# Autodesk Inventor assembly: bed
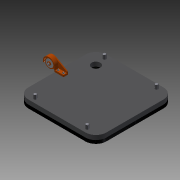
[picture p0: Inventor's stored thumbnail of the model, 180x180]
Saved by Autodesk Inventor 2013 (Build 170138000, 138)
## iProperties
Created: 2013-10-14
Part Number: bed
Document SubType Name: Assembly
Designer: employee
Author: employee
## Documents named in this file (13)
- C:\Users\employee\Desktop\ConceptFORGE\ConceptFORGE\Wally\bed.iam
- C:\Users\employee\Desktop\ConceptFORGE\ConceptFORGE\Wally\bed.ipt
- C:\Users\employee\Desktop\ConceptFORGE\ConceptFORGE\Wally\hot bed.ipt
- C:\Users\employee\Desktop\ConceptFORGE\ConceptFORGE\Wally\M3x16.ipt
- C:\Users\employee\Desktop\ConceptFORGE\ConceptFORGE\Wally\z pulley holder.ipt
- C:\Users\employee\Desktop\ConceptFORGE\ConceptFORGE\Wally\m3 nut.ipt
- C:\Users\employee\Desktop\ConceptFORGE\ConceptFORGE\Wally\608.ipt
- C:\Users\employee\Desktop\ConceptFORGE\ConceptFORGE\Wally\basalt.ipt
- C:\Users\employee\Desktop\ConceptFORGE\ConceptFORGE\Wally\M8x35.ipt
- C:\Users\employee\Desktop\ConceptFORGE\ConceptFORGE\Wally\plastic washer.ipt
- C:\Users\employee\Desktop\ConceptFORGE\ConceptFORGE\Wally\z idler.ipt
- C:\Users\employee\Desktop\ConceptFORGE\ConceptFORGE\Wally\z idler insert.ipt
- C:\Users\employee\Desktop\ConceptFORGE\ConceptFORGE\Wally\M3x14.ipt
## Components (21 placed, 11 different names)
1. bed:1 — Insert:1, Insert:2, Insert:3, Insert:11, Insert:12, Insert:22, Insert:23
2. hot bed:1 — Insert:3
3. Forged Socket Head Cap Screw - Metric M3x0.5 x 16:1 — Insert:1
4. Forged Socket Head Cap Screw - Metric M3x0.5 x 16:2 — Insert:2
5. z pulley holder:1 — Insert:22, Insert:23, Mate:1, Mate:2, Angle:1, Mate:3
6. Hex Nut Metric M3 x 0.5:1
7. Hex Nut Metric M3 x 0.5:2
8. Hex Nut Metric M3 x 0.5:3 — Mate:1, Mate:2, Angle:1
9. 608:1 — Insert:21, Mate:3, Insert:24
10. basalt:1 — Insert:11, Insert:12, Insert:13, Insert:14, Insert:15, Insert:16
11. Hex Bolt - Metric M8 x 1.25 x 35:1 — Insert:20
12. Hex Bolt - Metric M8 x 1.25 x 35:2 — Insert:19
13. Hex Bolt - Metric M8 x 1.25 x 35:3 — Insert:18
14. Hex Bolt - Metric M8 x 1.25 x 35:4 — Insert:17
15. plastic washer:1 — Insert:13, Insert:19
16. plastic washer:2 — Insert:14, Insert:18
17. plastic washer:3 — Insert:15, Insert:20
18. plastic washer:4 — Insert:16, Insert:17
19. z idler:1 — Insert:21
20. z idler insert:1 — Insert:24, Insert:25
21. Forged Socket Head Cap Screw - Metric M3x0.5 x 16:3 — Insert:25
## Relationships (22: Insert 18, Mate 3, Angle 1)
- Insert:1: bed:1 ↔ Forged Socket Head Cap Screw - Metric M3x0.5 x 16:1
- Insert:2: bed:1 ↔ Forged Socket Head Cap Screw - Metric M3x0.5 x 16:2
- Insert:3: bed:1 ↔ hot bed:1
- Insert:11: bed:1 ↔ basalt:1
- Insert:12: bed:1 ↔ basalt:1
- Insert:13: basalt:1 ↔ plastic washer:1
- Insert:14: basalt:1 ↔ plastic washer:2
- Insert:15: basalt:1 ↔ plastic washer:3
- Insert:16: basalt:1 ↔ plastic washer:4
- Insert:17: Hex Bolt - Metric M8 x 1.25 x 35:4 ↔ plastic washer:4
- Insert:18: Hex Bolt - Metric M8 x 1.25 x 35:3 ↔ plastic washer:2
- Insert:19: Hex Bolt - Metric M8 x 1.25 x 35:2 ↔ plastic washer:1
- Insert:20: Hex Bolt - Metric M8 x 1.25 x 35:1 ↔ plastic washer:3
- Insert:21: 608:1 ↔ z idler:1
- Insert:22: bed:1 ↔ z pulley holder:1
- Insert:23: bed:1 ↔ z pulley holder:1
- Mate:1: z pulley holder:1 ↔ Hex Nut Metric M3 x 0.5:3
- Mate:2: z pulley holder:1 ↔ Hex Nut Metric M3 x 0.5:3
- Angle:1 (0 deg): z pulley holder:1 ↔ Hex Nut Metric M3 x 0.5:3
- Mate:3: z pulley holder:1 ↔ 608:1
- Insert:24: 608:1 ↔ z idler insert:1
- Insert:25: z idler insert:1 ↔ Forged Socket Head Cap Screw - Metric M3x0.5 x 16:3
